# Autodesk Inventor assembly: Hinge
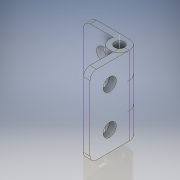
[picture p0: Inventor's stored thumbnail of the model, 180x180]
Saved by Autodesk Inventor 2016 (Build 200138000, 138)
## iProperties
Created: 2017-11-05
Part Number: Hinge
Document SubType Name: Assembly
Designer: mathaetaes
Author: mathaetaes
## Documents named in this file (3)
- E:\Projects\3D Printer\printer projects\My Designs\Bar Cabinet\Hinge.iam
- E:\Projects\3D Printer\printer projects\My Designs\Bar Cabinet\hinge left.ipt
- E:\Projects\3D Printer\printer projects\My Designs\Bar Cabinet\hinge right.ipt
## Components (2 placed, 2 different names)
1. hinge left:1 — Rotational:1
2. hinge right:1 — Rotational:1
## Relationships (1: RevoluteJoint 1)
- Rotational:1 [RevoluteJoint]: hinge left:1 ↔ hinge right:1
